# Autodesk Inventor assembly: gears
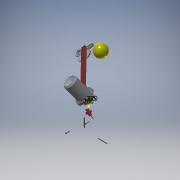
[picture p0: Inventor's stored thumbnail of the model, 180x180]
Saved by Autodesk Inventor 2019 (Build 230136000, 136)
## iProperties
Created: 2019-01-24
Part Number: gears
Document SubType Name: Assembly
Designer: Varga Daniel
Author: Varga Daniel
## Documents named in this file (14)
- C:\!_Dani\!_cloud\OneDrive\!_munka\Revolution\RevvyDemoKit\Structural parts\Part_test_Assembly.iam
- C:\!_Dani\!_cloud\OneDrive\!_munka\Revolution\RevvyDemoKit\Structural parts\Connetor Pins\Jasztool_old\cp1x1.ipt
- C:\!_Dani\!_cloud\OneDrive\!_munka\Revolution\RevvyDemoKit\Structural parts\Axle Connectors\Jasztool_old\Axle connector 3x3 cross.ipt
- C:\!_Dani\!_cloud\OneDrive\!_munka\Revolution\RevvyDemoKit\Structural parts\Gears\gear40.iam
- C:\!_Dani\!_cloud\OneDrive\!_munka\Revolution\RevvyDemoKit\Structural parts\Axles\Jasztool_old\Axle 2.ipt
- C:\!_Dani\!_cloud\OneDrive\!_munka\Revolution\RevvyDemoKit\Structural parts\Gears\gear60.iam
- C:\!_Dani\!_cloud\OneDrive\!_munka\Revolution\RevvyDemoKit\Structural parts\Axles\Jasztool_old\Axle 5s.ipt
- C:\!_Dani\!_cloud\OneDrive\!_munka\Revolution\RevvyDemoKit\Structural parts\Gears\gear20.iam
- C:\!_Dani\!_cloud\OneDrive\!_munka\Revolution\RevvyDemoKit\Structural parts\Gears\Gear_rack_8.ipt
- C:\!_Dani\!_cloud\OneDrive\!_munka\Revolution\RevvyDemoKit\Structural parts\Straight Beams\Jasztool_old\2x30.ipt
- C:\!_Dani\!_cloud\OneDrive\!_munka\Revolution\RevvyDemoKit\Structural parts\Curved beams\cocacola can.ipt
- C:\!_Dani\!_cloud\OneDrive\!_munka\Revolution\RevvyDemoKit\Structural parts\Curved beams\Tennis Ball.ipt
- C:\!_Dani\!_cloud\OneDrive\!_munka\Revolution\RevvyDemoKit\Structural parts\Curved beams\CB6H.ipt
- C:\!_Dani\!_cloud\OneDrive\!_munka\Revolution\RevvyDemoKit\Structural parts\Straight Beams\S2x1.iam
## Components (23 placed, 13 different names)
1. cp1x1:1 — Mate:3, Mate:4
2. gear40:1 [sub-assembly] — Mate:12, Mate:13, Flush:1, Mate:16, Mate:18, Mate:19, Mate:20
3. Axle connector 3x3 cross:2 — Mate:3, Mate:4
4. gear60:1 [sub-assembly] — Mate:10, Mate:11, Flush:2, Mate:17, Mate:18, Mate:22, Mate:26
5. Axle 2:3
6. Axle 2:4
7. cp1x1:2 — Mate:10, Mate:11
8. Axle 5s:1
9. Axle 5s:2 — Mate:12, Mate:13
10. gear20:1 [sub-assembly] — Mate:14, Mate:15, Flush:1, Mate:16, Flush:2, Mate:17
11. Axle 5s:3 — Mate:14, Mate:15
12. gear20:2 [sub-assembly] — Mate:19, Mate:20
13. Gear_rack_8:1 — Flush:3, Mate:24, Mate:25
14. 2x30:1 — Mate:22, Flush:3, Mate:24, Mate:25, Mate:26, Mate:27, Mate:28, Mate:29, Mate:30
15. cocacola can:1 — Mate:35, Mate:36, Flush:4, Mate:37
16. Tennis Ball:1
17. CB6H:1 — Mate:31, Mate:32, Mate:35, Flush:4, Flush:5, Mate:40
18. CB6H:2 — Mate:33, Mate:34, Mate:36
19. cp1x1:3 — Mate:27, Mate:28, Mate:31, Mate:32
20. cp1x1:4 — Mate:29, Mate:30, Mate:33, Mate:34
21. CB6H:3 — Mate:37, Flush:5, Mate:38, Mate:39, Mate:41, Mate:42
22. S2x1:1 [sub-assembly] — Mate:38, Mate:39, Mate:40
23. S2x1:2 [sub-assembly] — Mate:41, Mate:42
## Relationships (38: Mate 33, Flush 5)
- Mate:3: cp1x1:1 ↔ Axle connector 3x3 cross:2
- Mate:4: cp1x1:1 ↔ Axle connector 3x3 cross:2
- Mate:10: gear60:1 ↔ cp1x1:2
- Mate:11: gear60:1 ↔ cp1x1:2
- Mate:12: gear40:1 ↔ Axle 5s:2
- Mate:13: gear40:1 ↔ Axle 5s:2
- Mate:14: gear20:1 ↔ Axle 5s:3
- Mate:15: gear20:1 ↔ Axle 5s:3
- Flush:1: gear40:1 ↔ gear20:1
- Mate:16 (30 mm): gear40:1 ↔ gear20:1
- Flush:2: gear60:1 ↔ gear20:1
- Mate:17 (40 mm): gear60:1 ↔ gear20:1
- Mate:18 (50 mm): gear40:1 ↔ gear60:1
- Mate:19: gear40:1 ↔ gear20:2
- Mate:20: gear40:1 ↔ gear20:2
- Mate:22: gear60:1 ↔ 2x30:1
- Flush:3: Gear_rack_8:1 ↔ 2x30:1
- Mate:24: Gear_rack_8:1 ↔ 2x30:1
- Mate:25: Gear_rack_8:1 ↔ 2x30:1
- Mate:26: gear60:1 ↔ 2x30:1
- Mate:27: 2x30:1 ↔ cp1x1:3
- Mate:28: 2x30:1 ↔ cp1x1:3
- Mate:29: 2x30:1 ↔ cp1x1:4
- Mate:30: 2x30:1 ↔ cp1x1:4
- Mate:31: CB6H:1 ↔ cp1x1:3
- Mate:32: CB6H:1 ↔ cp1x1:3
- Mate:33: CB6H:2 ↔ cp1x1:4
- Mate:34: CB6H:2 ↔ cp1x1:4
- Mate:35: cocacola can:1 ↔ CB6H:1
- Mate:36: cocacola can:1 ↔ CB6H:2
- Flush:4 (-20 mm): cocacola can:1 ↔ CB6H:1
- Mate:37: cocacola can:1 ↔ CB6H:3
- Flush:5: CB6H:1 ↔ CB6H:3
- Mate:38: CB6H:3 ↔ S2x1:1
- Mate:39: CB6H:3 ↔ S2x1:1
- Mate:40: CB6H:1 ↔ S2x1:1
- Mate:41: CB6H:3 ↔ S2x1:2
- Mate:42: CB6H:3 ↔ S2x1:2
